# Autodesk Inventor assembly: CameraSetup
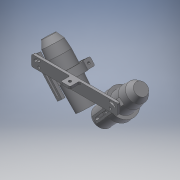
[picture p0: Inventor's stored thumbnail of the model, 180x180]
Saved by Autodesk Inventor 2019 (Build 230136000, 136)
## iProperties
Created: 2019-07-15
Part Number: CameraSetup
Document SubType Name: Assembly
Designer: aorfi
Author: aorfi
## Documents named in this file (5)
- C:\Users\aorfi\Documents\IQC\CameraSetup.iam
- C:\Users\aorfi\Documents\IQC\COTS\USBCamera.ipt
- C:\Users\aorfi\Documents\IQC\CustomParts\CameraClamp.ipt
- C:\Users\aorfi\Documents\IQC\CustomParts\CameraSlider.ipt
- C:\Users\aorfi\Documents\IQC\CustomParts\CameraBase.ipt
## Components (7 placed, 4 different names)
1. USBCamera:2 — Mate:2, Symmetry:1, Mate:10
2. CameraClamp:1 — Mate:1, Mate:3, Angle:1, Symmetry:2, Mate:11, Tangent:1
3. USBCamera:1 — Mate:1, Symmetry:1, Mate:11
4. CameraClamp:2 — Mate:2, Mate:5, Symmetry:2, Mate:10, Angle:2, Tangent:5
5. CameraSlider:1 — Mate:3, Angle:1, Mate:8, Tangent:1, Tangent:3, Symmetry:4
6. CameraSlider:2 — Mate:5, Mate:7, Symmetry:4, Tangent:4, Angle:2, Tangent:5
7. CameraBase:1 — Mate:7, Flush:1, Mate:8, Mate:12, Mate:14, Tangent:3, Tangent:4
## Relationships (20: Mate 10, Tangent 4, Symmetry 3, Angle 2, Flush 1)
- Mate:1: CameraClamp:1 ↔ USBCamera:1
- Mate:2: USBCamera:2 ↔ CameraClamp:2
- Mate:3: CameraClamp:1 ↔ CameraSlider:1
- Angle:1 (0 deg): CameraClamp:1 ↔ CameraSlider:1
- Mate:5: CameraClamp:2 ↔ CameraSlider:2
- Mate:7: CameraSlider:2 ↔ CameraBase:1
- Flush:1: CameraBase:1
- Mate:8: CameraSlider:1 ↔ CameraBase:1
- Symmetry:1: USBCamera:2 ↔ USBCamera:1
- Symmetry:2: CameraClamp:1 ↔ CameraClamp:2
- Mate:10: USBCamera:2 ↔ CameraClamp:2
- Mate:11: CameraClamp:1 ↔ USBCamera:1
- Mate:12: CameraBase:1
- Mate:14: CameraBase:1
- Tangent:1: CameraClamp:1 ↔ CameraSlider:1
- Tangent:3: CameraSlider:1 ↔ CameraBase:1
- Symmetry:4: CameraSlider:1 ↔ CameraSlider:2
- Tangent:4: CameraSlider:2 ↔ CameraBase:1
- Angle:2 (0 deg): CameraClamp:2 ↔ CameraSlider:2
- Tangent:5: CameraClamp:2 ↔ CameraSlider:2
